# Autodesk Inventor assembly: GoPlus
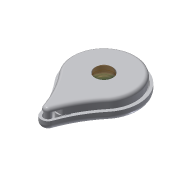
[picture p0: Inventor's stored thumbnail of the model, 180x180]
Saved by Autodesk Inventor 2016 SP1 (Build 200210100, 210)
## iProperties
Created: 2018-07-04
Part Number: GoPlus
Material: Generisch
Document SubType Name: Assembly
Designer: WhoTheHeck
Author: WhoTheHeck
## Documents named in this file (9)
- E:\Dokumente\PG+Ext\Modell\GoPlCase_v1\GoPlus.iam
- E:\Dokumente\PG+Ext\Modell\GoPlCase_v1\Button_plus.ipt
- E:\Dokumente\PG+Ext\Modell\GoPlCase_v1\rubberpad.ipt
- E:\Dokumente\PG+Ext\Modell\GoPlCase_v1\motor.ipt
- E:\Dokumente\PG+Ext\Modell\GoPlCase_v1\pcb.ipt
- E:\Dokumente\PG+Ext\Modell\GoPlCase_v1\top.ipt
- E:\Dokumente\PG+Ext\Modell\GoPlCase_v1\bot.ipt
- E:\Dokumente\PG+Ext\Modell\GoPlCase_v1\clamp_ring.ipt
- E:\Dokumente\PG+Ext\Modell\GoPlCase_v1\screw.ipt
## Components (8 placed, 8 different names)
1. Button_plus:1 — Passend:3, Passend:4, Passend:6, Passend:7
2. rubberpad:1 — Passend:3, Passend:4, Passend:8, Passend:9
3. motor:1 — Tangential:1, Passend:12, Tangential:2
4. pcb:1 — Passend:8, Passend:9, Passend:13
5. top:1 — Passend:6, Passend:7, Passend:10, Passend:11, Tangential:1, Passend:12, Tangential:2, Passend:13, Passend:14, Passend:15
6. bot:1 — Passend:14, Passend:15, Passend:16, Passend:17, Passend:18, Passend:19
7. clamp_ring:1 — Passend:16, Passend:17
8. screw:1 — Passend:18, Passend:19
## Relationships (18: Mate 16, Tangent 2)
- Passend:3 [Mate]: Button_plus:1 ↔ rubberpad:1
- Passend:4 [Mate]: Button_plus:1 ↔ rubberpad:1
- Passend:6 [Mate]: Button_plus:1 ↔ top:1
- Passend:7 [Mate]: Button_plus:1 ↔ top:1
- Passend:8 [Mate]: rubberpad:1 ↔ pcb:1
- Passend:9 [Mate]: rubberpad:1 ↔ pcb:1
- Passend:10 [Mate]: top:1
- Passend:11 [Mate]: top:1
- Tangential:1: motor:1 ↔ top:1
- Passend:12 [Mate] (0.5 mm): motor:1 ↔ top:1
- Tangential:2: motor:1 ↔ top:1
- Passend:13 [Mate]: pcb:1 ↔ top:1
- Passend:14 [Mate]: top:1 ↔ bot:1
- Passend:15 [Mate]: top:1 ↔ bot:1
- Passend:16 [Mate]: bot:1 ↔ clamp_ring:1
- Passend:17 [Mate]: bot:1 ↔ clamp_ring:1
- Passend:18 [Mate]: bot:1 ↔ screw:1
- Passend:19 [Mate]: bot:1 ↔ screw:1
